# Autodesk Inventor assembly: Сборка всего
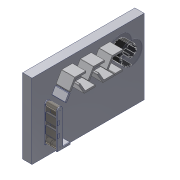
[picture p0: Inventor's stored thumbnail of the model, 180x180]
Saved by Autodesk Inventor 2022 (Build 260153000, 153)
## iProperties
Created: 2023-02-18
Part Number: Сборка всего
Document SubType Name: Assembly
Designer: Глеб
Mass: 12847.1 g
Surface Area: 9212.86 cm^2
Volume: 12847.1 cm^3
Density: 1 g/cm^3
Author: Глеб
## Documents named in this file (6)
- C:\Users\Глеб\Documents\Inventor\Файлы Inventor\Сборка всего.iam
- C:\Users\Глеб\Documents\Inventor\Файлы Inventor\Общий концепт в 3д.ipt
- C:\Users\Глеб\Documents\Inventor\Файлы Inventor\Барабан сборка.iam
- C:\Users\Глеб\Documents\Inventor\Файлы Inventor\Лепестки со шпильками сборка.iam
- C:\Users\Глеб\Documents\Inventor\Файлы Inventor\Конвейр сборка.iam
- C:\Users\Глеб\Documents\Inventor\Файлы Inventor\Стенка БСП.iam
## Components (11 placed, 5 different names)
1. Общий концепт в 3д:1 — Совмещение:47, Совмещение:48, Заподлицо:12, Совмещение:52, Совмещение:53, Совмещение:56
2. Барабан сборка:1 [sub-assembly] — Совмещение:47, Совмещение:50, Совмещение:51
3. Лепестки со шпильками сборка:1 [sub-assembly] — Угол:1, Угол:2, Совмещение:48, Заподлицо:1, Заподлицо:4, Заподлицо:6, Заподлицо:7, Совмещение:49, Заподлицо:8, Заподлицо:12, Симметрия:1
4. Лепестки со шпильками сборка:5 [sub-assembly] — Угол:3, Угол:4, Заподлицо:2, Заподлицо:7, Совмещение:49, Заподлицо:8, Заподлицо:9, Симметрия:1, Заподлицо:14, Совмещение:54
5. Конвейр сборка:1 [sub-assembly] — Совмещение:56
6. Лепестки со шпильками сборка:6 [sub-assembly] — Заподлицо:1, Заподлицо:3, Заподлицо:5, Заподлицо:9, Заподлицо:10
7. Лепестки со шпильками сборка:7 [sub-assembly] — Заподлицо:2, Заподлицо:6, Заподлицо:10, Заподлицо:11
8. Лепестки со шпильками сборка:8 [sub-assembly] — Заподлицо:3, Заподлицо:4, Заподлицо:5, Заподлицо:11, Заподлицо:15, Совмещение:55
9. Стенка БСП:1 [sub-assembly] — Заподлицо:14, Совмещение:52, Совмещение:54, Заподлицо:16, Заподлицо:17, Угол:5
10. Стенка БСП:2 [sub-assembly] — Заподлицо:15, Совмещение:53, Совмещение:55
11. Стенка БСП:3 [sub-assembly] — Заподлицо:17, Угол:5
## Relationships (33: Flush 17, Mate 10, Angle 5, Symmetry 1)
- Совмещение:47 [Mate]: Общий концепт в 3д:1 ↔ Барабан сборка:1
- Угол:1 [Angle] (0 deg): Лепестки со шпильками сборка:1
- Угол:2 [Angle] (0 deg): Лепестки со шпильками сборка:1
- Совмещение:48 [Mate]: Общий концепт в 3д:1 ↔ Лепестки со шпильками сборка:1
- Угол:3 [Angle] (0 deg): Лепестки со шпильками сборка:5
- Угол:4 [Angle] (180 deg): Лепестки со шпильками сборка:5
- Заподлицо:1 [Flush]: Лепестки со шпильками сборка:1 ↔ Лепестки со шпильками сборка:6
- Заподлицо:2 [Flush]: Лепестки со шпильками сборка:5 ↔ Лепестки со шпильками сборка:7
- Заподлицо:3 [Flush]: Лепестки со шпильками сборка:6 ↔ Лепестки со шпильками сборка:8
- Заподлицо:4 [Flush]: Лепестки со шпильками сборка:1 ↔ Лепестки со шпильками сборка:8
- Заподлицо:5 [Flush]: Лепестки со шпильками сборка:6 ↔ Лепестки со шпильками сборка:8
- Заподлицо:6 [Flush]: Лепестки со шпильками сборка:1 ↔ Лепестки со шпильками сборка:7
- Заподлицо:7 [Flush]: Лепестки со шпильками сборка:1 ↔ Лепестки со шпильками сборка:5
- Совмещение:49 [Mate] (-100 mm): Лепестки со шпильками сборка:1 ↔ Лепестки со шпильками сборка:5
- Заподлицо:8 [Flush] (-50 mm): Лепестки со шпильками сборка:1 ↔ Лепестки со шпильками сборка:5
- Заподлицо:9 [Flush] (-50 mm): Лепестки со шпильками сборка:5 ↔ Лепестки со шпильками сборка:6
- Заподлицо:10 [Flush] (-50 mm): Лепестки со шпильками сборка:6 ↔ Лепестки со шпильками сборка:7
- Заподлицо:11 [Flush] (-50 mm): Лепестки со шпильками сборка:7 ↔ Лепестки со шпильками сборка:8
- Заподлицо:12 [Flush] (40 mm): Общий концепт в 3д:1 ↔ Лепестки со шпильками сборка:1
- Симметрия:1 [Symmetry]: Лепестки со шпильками сборка:1 ↔ Лепестки со шпильками сборка:5
- Совмещение:50 [Mate]: Барабан сборка:1
- Заподлицо:13 [Flush] (-14 mm)
- Совмещение:51 [Mate]: Барабан сборка:1
- Заподлицо:14 [Flush]: Лепестки со шпильками сборка:5 ↔ Стенка БСП:1
- Совмещение:52 [Mate]: Общий концепт в 3д:1 ↔ Стенка БСП:1
- Заподлицо:15 [Flush]: Лепестки со шпильками сборка:8 ↔ Стенка БСП:2
- Совмещение:53 [Mate]: Общий концепт в 3д:1 ↔ Стенка БСП:2
- Совмещение:54 [Mate] (5 mm): Лепестки со шпильками сборка:5 ↔ Стенка БСП:1
- Совмещение:55 [Mate] (5 mm): Лепестки со шпильками сборка:8 ↔ Стенка БСП:2
- Заподлицо:16 [Flush] (70 mm): Стенка БСП:1
- Совмещение:56 [Mate]: Общий концепт в 3д:1 ↔ Конвейр сборка:1
- Заподлицо:17 [Flush]: Стенка БСП:1 ↔ Стенка БСП:3
- Угол:5 [Angle] (30 deg): Стенка БСП:1 ↔ Стенка БСП:3
